# Autodesk Inventor assembly: frame_bottom
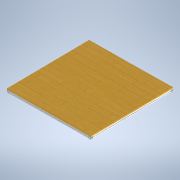
[picture p0: Inventor's stored thumbnail of the model, 180x180]
Saved by Autodesk Inventor 2021.3 (Build 253353000, 353)
## iProperties
Created: 2023-04-06
Part Number: frame_bottom
Document SubType Name: Assembly
Designer: nxf77172
_SolveAssemblyDoc: Frame Generator Solve Assembly
_Version: 15.0.0
Author: nxf77172
## Documents named in this file (5)
- C:\Users\nxf77172\Desktop\mechanical_cleaned\custom_parts\frame\frame_top.iam
- C:\Users\nxf77172\Desktop\mechanical_cleaned\custom_parts\frame\frame_outline.ipt
- C:\Users\nxf77172\Desktop\mechanical_cleaned\custom_parts\aluminium profile\angle_connector_x3.ipt
- C:\Users\nxf77172\Desktop\mechanical_cleaned\custom_parts\frame\frame_top\Frame\Frame 1683900195586.iam
- C:\Users\nxf77172\Desktop\mechanical_cleaned\custom_parts\Top_Plate.ipt
## Components (7 placed, 4 different names)
1. frame_outline:1 — Flush:2, Mate:2
2. Frame 1683900195586:1 [sub-assembly] — Mate:3, Mate:4, Flush:3, Mate:5, Mate:6, Flush:4, Mate:7, Mate:8, Flush:5, Mate:9, Mate:10, Flush:6, Mate:11, Flush:7, Flush:8
3. angle_connector_x3:1 — Mate:3, Mate:4, Flush:3
4. angle_connector_x3:2 — Mate:5, Mate:6, Flush:4
5. angle_connector_x3:3 — Mate:7, Mate:8, Flush:5
6. angle_connector_x3:4 — Mate:9, Mate:10, Flush:6
7. Top_Plate:1 — Mate:11, Flush:7, Flush:8
## Relationships (17: Mate 10, Flush 7)
- Flush:2: frame_outline:1
- Mate:2: frame_outline:1
- Mate:3: Frame 1683900195586:1 ↔ angle_connector_x3:1
- Mate:4: Frame 1683900195586:1 ↔ angle_connector_x3:1
- Flush:3: Frame 1683900195586:1 ↔ angle_connector_x3:1
- Mate:5: Frame 1683900195586:1 ↔ angle_connector_x3:2
- Mate:6: Frame 1683900195586:1 ↔ angle_connector_x3:2
- Flush:4: Frame 1683900195586:1 ↔ angle_connector_x3:2
- Mate:7: Frame 1683900195586:1 ↔ angle_connector_x3:3
- Mate:8: Frame 1683900195586:1 ↔ angle_connector_x3:3
- Flush:5: Frame 1683900195586:1 ↔ angle_connector_x3:3
- Mate:9: Frame 1683900195586:1 ↔ angle_connector_x3:4
- Mate:10: Frame 1683900195586:1 ↔ angle_connector_x3:4
- Flush:6: Frame 1683900195586:1 ↔ angle_connector_x3:4
- Mate:11: Frame 1683900195586:1 ↔ Top_Plate:1
- Flush:7: Frame 1683900195586:1 ↔ Top_Plate:1
- Flush:8: Frame 1683900195586:1 ↔ Top_Plate:1
